# Autodesk Inventor assembly: final assembly
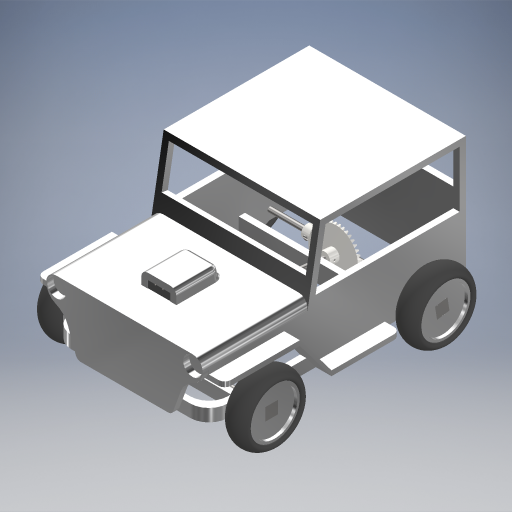
[picture p0: Inventor's stored thumbnail of the model, 512x512]
Saved by Autodesk Inventor 2024 (Build 280153000, 153)
## iProperties
Created: 2024-04-13
Part Number: final assembly
Document SubType Name: Assembly
Designer: Alex
Author: Alex
## Documents named in this file (12)
- C:\Shared\alex-bartella-schoolwork\4z03\final\final\final assembly.iam
- C:\Shared\alex-bartella-schoolwork\4z03\final\rear axle.ipt
- C:\Shared\alex-bartella-schoolwork\4z03\final\final\gears\Bevel Gear14.ipt
- C:\Shared\alex-bartella-schoolwork\4z03\final\shell.ipt
- C:\Shared\alex-bartella-schoolwork\4z03\final\final\wheel.iam
- C:\Shared\alex-bartella-schoolwork\4z03\final\front axle.ipt
- C:\Shared\alex-bartella-schoolwork\4z03\final\rc_motor\rc_motor.ipt
- C:\Shared\alex-bartella-schoolwork\4z03\final\driveshaft.ipt
- C:\Shared\alex-bartella-schoolwork\4z03\final\final\gears\Bevel Gear24.ipt
- C:\Shared\alex-bartella-schoolwork\4z03\final\rc_battery\rc_battery.ipt
- C:\Users\turbo\Documents\Inventor\Content Center Files\R2024\en-US\ANSI_ASME B18.6.5M(1)\ANSI_ASME B18.6.5M - M3x0.5 x 6(1) T.ipt
- C:\Users\turbo\Documents\Inventor\Content Center Files\R2024\en-US\ANSI_ASME B18.6.5M(1)\ANSI_ASME B18.6.5M - M3.5x0.6 x 20(1) T.ipt
## Components (20 placed, 11 different names)
1. shell:1 — Flush:1, Flush:2, Flush:3, Mate:3, Mate:4, Mate:6, Mate:8, Mate:13, Mate:15, Mate:17, Mate:18, Angle:1, Mate:21, Mate:23, Mate:24, Mate:25, Mate:26, Angle:3, Mate:27, Angle:4, Mate:28, Angle:5
2. rear axle:1 — Mate:1, Mate:2, Mate:3, Mate:11, Mate:12, Mate:14, Mate:16
3. Bevel Gear1:1 — Mate:1, Mate:2, Rotation:1, Mate:36
4. wheel:1 [sub-assembly] — Mate:5, Mate:6, Mate:10
5. wheel:2 [sub-assembly] — Mate:7, Mate:8, Mate:9
6. wheel:3 [sub-assembly] — Mate:11, Mate:13, Mate:14
7. wheel:4 [sub-assembly] — Mate:12, Mate:15, Mate:16
8. front axle:1 — Mate:4, Mate:5, Mate:7, Mate:9, Mate:10
9. rc_motor:1 — Mate:17, Mate:18, Angle:1, Mate:22, Driver, Mate:29, Mate:30, Mate:31, Mate:32, Mate:33, Mate:34
10. driveshaft:1 — Mate:19, Flush:4, Mate:20, Mate:21, Mate:22, Driver
11. Bevel Gear2:1 — Mate:19, Flush:4, Mate:20, Rotation:1, Mate:35
12. rc_battery:1 — Mate:23, Mate:24, Mate:25
13. Slotted Flat Countersunk Head Tapping Screw - Type T - Metric M3x0.5 x 6:1 — Mate:29
14. Slotted Flat Countersunk Head Tapping Screw - Type T - Metric M3x0.5 x 6:2 — Mate:30
15. Slotted Flat Countersunk Head Tapping Screw - Type T - Metric M3x0.5 x 6:3 — Mate:31
16. Slotted Flat Countersunk Head Tapping Screw - Type T - Metric M3x0.5 x 6:4 — Mate:32
17. Slotted Flat Countersunk Head Tapping Screw - Type T - Metric M3x0.5 x 6:5 — Mate:33
18. Slotted Flat Countersunk Head Tapping Screw - Type T - Metric M3x0.5 x 6:6 — Mate:34
19. Slotted Flat Countersunk Head Tapping Screw - Type T - Metric M3.5x0.6 x 20:1 — Mate:35
20. Slotted Flat Countersunk Head Tapping Screw - Type T - Metric M3.5x0.6 x 20:2 — Mate:36
## Relationships (49: Mate 36, Flush 6, Angle 5, RelateRotation 1, Symmetry 1)
- Mate:1: rear axle:1 ↔ Bevel Gear1:1
- Mate:2: rear axle:1 ↔ Bevel Gear1:1
- Flush:1: shell:1
- Flush:2: shell:1
- Flush:3: shell:1
- Mate:3: shell:1 ↔ rear axle:1
- Mate:4: shell:1 ↔ front axle:1
- Mate:5: wheel:1 ↔ front axle:1
- Mate:6: shell:1 ↔ wheel:1
- Mate:7: wheel:2 ↔ front axle:1
- Mate:8: shell:1 ↔ wheel:2
- Mate:9: wheel:2 ↔ front axle:1
- Mate:10: wheel:1 ↔ front axle:1
- Mate:11: rear axle:1 ↔ wheel:3
- Mate:12: rear axle:1 ↔ wheel:4
- Mate:13: shell:1 ↔ wheel:3
- Mate:14: rear axle:1 ↔ wheel:3
- Mate:15: shell:1 ↔ wheel:4
- Mate:16: rear axle:1 ↔ wheel:4
- Mate:17: shell:1 ↔ rc_motor:1
- Mate:18: shell:1 ↔ rc_motor:1
- Angle:1 (0 deg): shell:1 ↔ rc_motor:1
- Mate:19: driveshaft:1 ↔ Bevel Gear2:1
- Flush:4: driveshaft:1 ↔ Bevel Gear2:1
- Mate:20: driveshaft:1 ↔ Bevel Gear2:1
- Mate:21: shell:1 ↔ driveshaft:1
- Mate:22: rc_motor:1 ↔ driveshaft:1
- Rotation:1 [RelateRotation] (3.3333 ul): Bevel Gear1:1 ↔ Bevel Gear2:1
- Mate:23: shell:1 ↔ rc_battery:1
- Mate:24: shell:1 ↔ rc_battery:1
- Mate:25: shell:1 ↔ rc_battery:1
- Driver [Angle] (0 deg): rc_motor:1 ↔ driveshaft:1
- Mate:26: shell:1
- Angle:3 (-6 deg): shell:1
- Flush:5 (3.211 mm)
- Flush:6 (5 mm)
- Mate:27: shell:1
- Angle:4 (0 deg): shell:1
- Mate:28: shell:1
- Angle:5 (0 deg): shell:1
- Symmetry:1
- Mate:29: rc_motor:1 ↔ Slotted Flat Countersunk Head Tapping Screw - Type T - Metric M3x0.5 x 6:1
- Mate:30: rc_motor:1 ↔ Slotted Flat Countersunk Head Tapping Screw - Type T - Metric M3x0.5 x 6:2
- Mate:31: rc_motor:1 ↔ Slotted Flat Countersunk Head Tapping Screw - Type T - Metric M3x0.5 x 6:3
- Mate:32: rc_motor:1 ↔ Slotted Flat Countersunk Head Tapping Screw - Type T - Metric M3x0.5 x 6:4
- Mate:33: rc_motor:1 ↔ Slotted Flat Countersunk Head Tapping Screw - Type T - Metric M3x0.5 x 6:5
- Mate:34: rc_motor:1 ↔ Slotted Flat Countersunk Head Tapping Screw - Type T - Metric M3x0.5 x 6:6
- Mate:35: Bevel Gear2:1 ↔ Slotted Flat Countersunk Head Tapping Screw - Type T - Metric M3.5x0.6 x 20:1
- Mate:36: Bevel Gear1:1 ↔ Slotted Flat Countersunk Head Tapping Screw - Type T - Metric M3.5x0.6 x 20:2
